# Autodesk Inventor assembly: LiftAssembly_Through
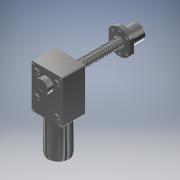
[picture p0: Inventor's stored thumbnail of the model, 180x180]
Saved by Autodesk Inventor 2018 (Build 220112000, 112)
## iProperties
Created: 2018-04-10
Part Number: LiftAssembly_Through
Document SubType Name: Assembly
Designer: P136265
Author: P136265
## Documents named in this file (6)
- C:\Users\P136265\Documents\GitHub\mecanum-cad\LiftAssembly_Through.iam
- C:\Users\P136265\Documents\GitHub\mecanum-cad\TS-58GZ868D_Open.ipt
- C:\Users\P136265\Documents\Inventor\Content Center Files\R2018\en-US\ISO 3031(1)\ISO 3031 - 12 x 26 x 2(1).ipt
- C:\Users\P136265\Documents\GitHub\mecanum-cad\ThrustWasher.ipt
- C:\Users\P136265\Documents\GitHub\mecanum-cad\12mm Ball Screw.ipt
- C:\Users\P136265\Documents\GitHub\mecanum-cad\16mm Lead Nut.ipt
## Components (6 placed, 5 different names)
1. TS-58GZ868D_Open:1 — Mate:14, Angle:2, Mate:16, Mate:24, Flush:2, Mate:27, Angle:3
2. ISO 3031Thrust Needle Roller And Cage Assembly 12 x 26 x 2:1 — Mate:21, Mate:22, Mate:23
3. ThrustWasher:1 — Mate:22, Mate:23, Mate:26
4. ThrustWasher:2 — Mate:21, Mate:25, Mate:26
5. 12mm Ball Screw:1 — Mate:24, Mate:25, Flush:2, Flush:3
6. 16mm Lead Nut:1 — Mate:27, Flush:3, Angle:3
## Relationships (13: Mate 9, Angle 2, Flush 2)
- Mate:14: TS-58GZ868D_Open:1
- Angle:2 (0 deg): TS-58GZ868D_Open:1
- Mate:16: TS-58GZ868D_Open:1
- Mate:21 (0.2 mm): ISO 3031Thrust Needle Roller And Cage Assembly 12 x 26 x 2:1 ↔ ThrustWasher:2
- Mate:22: ISO 3031Thrust Needle Roller And Cage Assembly 12 x 26 x 2:1 ↔ ThrustWasher:1
- Mate:23 (0.2 mm): ISO 3031Thrust Needle Roller And Cage Assembly 12 x 26 x 2:1 ↔ ThrustWasher:1
- Mate:24: TS-58GZ868D_Open:1 ↔ 12mm Ball Screw:1
- Mate:25: ThrustWasher:2 ↔ 12mm Ball Screw:1
- Mate:26: ThrustWasher:1 ↔ ThrustWasher:2
- Flush:2 (-130 mm): TS-58GZ868D_Open:1 ↔ 12mm Ball Screw:1
- Mate:27: TS-58GZ868D_Open:1 ↔ 16mm Lead Nut:1
- Flush:3: 12mm Ball Screw:1 ↔ 16mm Lead Nut:1
- Angle:3 (0 deg): TS-58GZ868D_Open:1 ↔ 16mm Lead Nut:1
